# Autodesk Inventor assembly: kolo_MIR
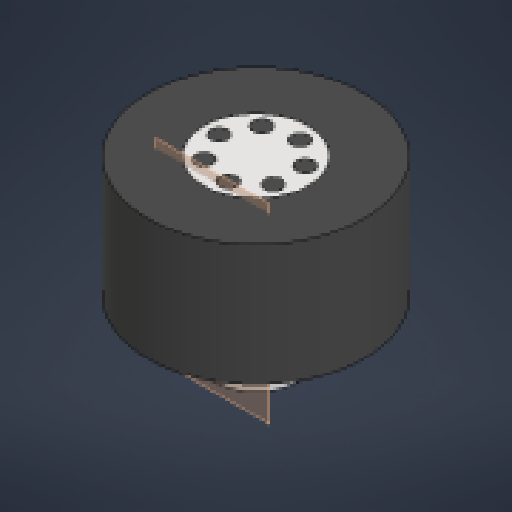
[picture p0: Inventor's stored thumbnail of the model, 512x512]
Saved by Autodesk Inventor 2023 (Build 270158000, 158)
## iProperties
Created: 2024-03-01
Part Number: kolo_MIR
Document SubType Name: Assembly
Designer: Michał
Author: Michał
## Documents named in this file (3)
- D:\Projekty\Roboilo\Ser\3D\3D\V2\Naped\kolo_MIR.iam
- D:\Projekty\Roboilo\Ser\3D\3D\V2\Naped\kolo\felga_MIR.ipt
- D:\Projekty\Roboilo\Ser\3D\3D\V2\Naped\kolo\opona_MIR.ipt
## Components (2 placed, 2 different names)
1. felga_MIR:1 — Flush:1
2. opona_MIR:1 — Flush:1
## Relationships (1: Mate 1)
- Flush:1 [Mate]: felga_MIR:1 ↔ opona_MIR:1
